# Autodesk Inventor assembly: MultiPassSCAN_outsideIn-DFMOD
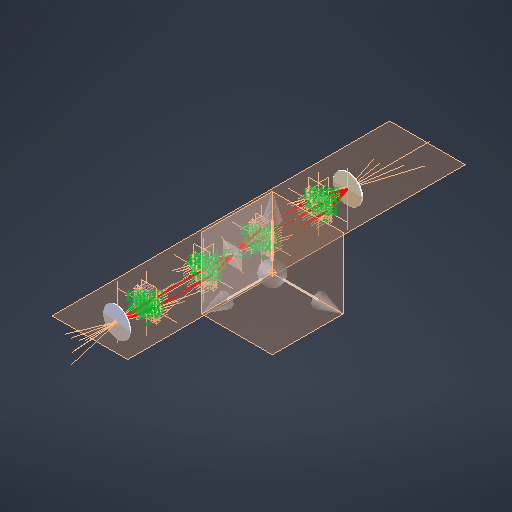
[picture p0: Inventor's stored thumbnail of the model, 512x512]
Saved by Autodesk Inventor 2026.1 (Build 301233000, 233)
## iProperties
Created: 2024-08-19
Part Number: MultiPassSCAN_outsideIn-DFMOD
Document SubType Name: Assembly
Designer: User
Author: User
## Documents named in this file (15)
- C:\Users\farin012\Downloads\fig4\fig4\MultiPassSCAN_outsideIn-DFMOD.iam
- C:\Users\farin012\Downloads\fig4\fig4\BB1-E02-Solidworks.ipt
- C:\Users\farin012\Downloads\fig4\fig4\LaserBeamEntry2.ipt
- C:\Users\farin012\Downloads\fig4\fig4\LoopPlane1.ipt
- C:\Users\farin012\Downloads\fig4\fig4\LA1608-AB-Solidworks\LA1608-AB-2LOOP_grid.ipt
- C:\Users\farin012\Downloads\fig4\fig4\LOOP1_COLL.ipt
- C:\Users\farin012\Downloads\fig4\fig4\LOOP1_COLL_PREDEF1.ipt
- C:\Users\farin012\Downloads\fig4\fig4\LOOP1_COLL_POSTDEF1.ipt
- C:\Users\farin012\Downloads\fig4\fig4\deflection_plane.ipt
- C:\Users\farin012\Downloads\fig4\fig4\LOOP1_COLL_PREDEF2.ipt
- C:\Users\farin012\Downloads\fig4\fig4\LOOP1_COLL_POSTDEF2.ipt
- C:\Users\farin012\Downloads\fig4\fig4\LOOP2_COLL_PREDEF1.ipt
- C:\Users\farin012\Downloads\fig4\fig4\LOOP2_COLL_POSTDEF1.ipt
- C:\Users\farin012\Downloads\fig4\fig4\LOOP2_COLL_PREDEF2.ipt
- C:\Users\farin012\Downloads\fig4\fig4\LOOP2_COLL_POSTDEF2.ipt
## Components (40 placed, 14 different names)
1. BB1-E02-Solidworks:1 — Mate:115, Mate:125, Mate:126, Mate:127, Angle:6, Mate:128, Mate:147
2. BB1-E02-Solidworks:2 — Angle:5, Mate:137, Mate:138
3. LaserBeamEntry2:16 — Mate:124, Flush:7
4. LoopPlane1:1 — Mate:113
5. LA1608-AB-2LOOP_grid:1 — Flush:3, Mate:124, Flush:7, Flush:8, Mate:129, Mate:145, Mate:147, Mate:148, Mate:172, Flush:164, Mate:173, Mate:174, Mate:175, Mate:176, Mate:177, Flush:165
6. LA1608-AB-2LOOP_grid:2 — Flush:2, Flush:9, Mate:130, Mate:145, Mate:146, Mate:149, Mate:154, Mate:155, Mate:156, Mate:169, Mate:170, Mate:171, Flush:163, Mate:178, Flush:166, Mate:179, Mate:180, Mate:193, Mate:194, Mate:195, Flush:171
7. LA1608-AB-2LOOP_grid:3 — Flush:5, Mate:137, Mate:151, Mate:152, Mate:160, Flush:160, Mate:161, Mate:162, Mate:163, Mate:164, Mate:165, Flush:161, Mate:184, Flush:168, Mate:185, Mate:186, Mate:187, Mate:188, Mate:189, Flush:169
8. LA1608-AB-2LOOP_grid:4 — Flush:4, Mate:146, Mate:150, Mate:152, Mate:159, Flush:159, Mate:166, Flush:162, Mate:167, Mate:168, Mate:181, Mate:182, Mate:183, Flush:167, Mate:190, Flush:170, Mate:191, Mate:192
9. LOOP1_COLL:1 — Mate:125, Mate:126
10. LOOP1_COLL:2 — Mate:127, Mate:128
11. LaserBeamEntry2:17 — Flush:8, Mate:129
12. LaserBeamEntry2:18 — Flush:9, Mate:130
13. LOOP1_COLL_PREDEF1:1 — Mate:155, Mate:156
14. LOOP1_COLL_POSTDEF1:1 — Mate:157, Mate:158
15. deflection_plane:1 — Mate:153, Mate:154, Flush:158, Mate:157, Mate:158
16. LaserBeamEntry2:19 — Mate:159, Flush:159
17. LaserBeamEntry2:20 — Mate:160, Flush:160
18. LOOP1_COLL_POSTDEF1:2 — Mate:161, Mate:162
19. LOOP1_COLL_POSTDEF1:3 — Mate:163, Mate:164
20. LaserBeamEntry2:21 — Mate:166, Flush:162
21. LaserBeamEntry2:22 — Mate:165, Flush:161
22. LOOP1_COLL_PREDEF2:1 — Mate:167, Mate:168
23. LOOP1_COLL_POSTDEF2:1 — Mate:169, Mate:170
24. LaserBeamEntry2:23 — Mate:172, Flush:164
25. LaserBeamEntry2:24 — Mate:171, Flush:163
26. LOOP2_COLL_PREDEF1:1 — Mate:173, Mate:174
27. LOOP2_COLL_PREDEF1:2 — Mate:175, Mate:176
28. LaserBeamEntry2:25 — Mate:177, Flush:165
29. LaserBeamEntry2:26 — Mate:178, Flush:166
30. LOOP2_COLL_PREDEF1:3 — Mate:179, Mate:180
31. LOOP2_COLL_POSTDEF1:1 — Mate:181, Mate:182
32. LaserBeamEntry2:27 — Mate:184, Flush:168
33. LaserBeamEntry2:28 — Mate:183, Flush:167
34. LOOP2_COLL_POSTDEF1:2 — Mate:185, Mate:186
35. LOOP2_COLL_PREDEF2:1 — Mate:187, Mate:188
36. LaserBeamEntry2:29 — Mate:189, Flush:169
37. LaserBeamEntry2:30 — Mate:190, Flush:170
38. LOOP2_COLL_PREDEF2:2 — Mate:191, Mate:192
39. LOOP2_COLL_POSTDEF2:1 — Mate:193, Mate:194
40. LaserBeamEntry2:31 — Mate:195, Flush:171
## Relationships (87: Mate 64, Flush 21, Angle 2)
- Mate:22
- Mate:23
- Mate:113: LoopPlane1:1
- Mate:115: BB1-E02-Solidworks:1
- Angle:5 (180 deg): BB1-E02-Solidworks:2
- Flush:2: LA1608-AB-2LOOP_grid:2
- Flush:3: LA1608-AB-2LOOP_grid:1
- Flush:4: LA1608-AB-2LOOP_grid:4
- Flush:5: LA1608-AB-2LOOP_grid:3
- Mate:124: LaserBeamEntry2:16 ↔ LA1608-AB-2LOOP_grid:1
- Flush:7: LaserBeamEntry2:16 ↔ LA1608-AB-2LOOP_grid:1
- Mate:125: BB1-E02-Solidworks:1 ↔ LOOP1_COLL:1
- Mate:126: BB1-E02-Solidworks:1 ↔ LOOP1_COLL:1
- Mate:127: BB1-E02-Solidworks:1 ↔ LOOP1_COLL:2
- Angle:6 (0 deg): BB1-E02-Solidworks:1
- Mate:128: BB1-E02-Solidworks:1 ↔ LOOP1_COLL:2
- Flush:8: LA1608-AB-2LOOP_grid:1 ↔ LaserBeamEntry2:17
- Mate:129: LA1608-AB-2LOOP_grid:1 ↔ LaserBeamEntry2:17
- Flush:9: LA1608-AB-2LOOP_grid:2 ↔ LaserBeamEntry2:18
- Mate:130: LA1608-AB-2LOOP_grid:2 ↔ LaserBeamEntry2:18
- Mate:137 (25 mm): BB1-E02-Solidworks:2 ↔ LA1608-AB-2LOOP_grid:3
- Mate:138: BB1-E02-Solidworks:2
- Mate:145 (-50 mm): LA1608-AB-2LOOP_grid:1 ↔ LA1608-AB-2LOOP_grid:2
- Mate:146 (50 mm): LA1608-AB-2LOOP_grid:2 ↔ LA1608-AB-2LOOP_grid:4
- Mate:147 (25 mm): BB1-E02-Solidworks:1 ↔ LA1608-AB-2LOOP_grid:1
- Mate:148: LA1608-AB-2LOOP_grid:1
- Mate:149: LA1608-AB-2LOOP_grid:2
- Mate:150: LA1608-AB-2LOOP_grid:4
- Mate:151: LA1608-AB-2LOOP_grid:3
- Mate:152 (-50 mm): LA1608-AB-2LOOP_grid:3 ↔ LA1608-AB-2LOOP_grid:4
- Mate:153: deflection_plane:1
- Mate:154 (25 mm): LA1608-AB-2LOOP_grid:2 ↔ deflection_plane:1
- Mate:155: LA1608-AB-2LOOP_grid:2 ↔ LOOP1_COLL_PREDEF1:1
- Mate:156: LA1608-AB-2LOOP_grid:2 ↔ LOOP1_COLL_PREDEF1:1
- Flush:158: deflection_plane:1
- Mate:157: LOOP1_COLL_POSTDEF1:1 ↔ deflection_plane:1
- Mate:158: LOOP1_COLL_POSTDEF1:1 ↔ deflection_plane:1
- Mate:159: LA1608-AB-2LOOP_grid:4 ↔ LaserBeamEntry2:19
- Flush:159: LA1608-AB-2LOOP_grid:4 ↔ LaserBeamEntry2:19
- Mate:160: LA1608-AB-2LOOP_grid:3 ↔ LaserBeamEntry2:20
- Flush:160: LA1608-AB-2LOOP_grid:3 ↔ LaserBeamEntry2:20
- Mate:161: LA1608-AB-2LOOP_grid:3 ↔ LOOP1_COLL_POSTDEF1:2
- Mate:162: LA1608-AB-2LOOP_grid:3 ↔ LOOP1_COLL_POSTDEF1:2
- Mate:163: LA1608-AB-2LOOP_grid:3 ↔ LOOP1_COLL_POSTDEF1:3
- Mate:164: LA1608-AB-2LOOP_grid:3 ↔ LOOP1_COLL_POSTDEF1:3
- Mate:165: LA1608-AB-2LOOP_grid:3 ↔ LaserBeamEntry2:22
- Flush:161: LA1608-AB-2LOOP_grid:3 ↔ LaserBeamEntry2:22
- Mate:166: LA1608-AB-2LOOP_grid:4 ↔ LaserBeamEntry2:21
- Flush:162: LA1608-AB-2LOOP_grid:4 ↔ LaserBeamEntry2:21
- Mate:167: LA1608-AB-2LOOP_grid:4 ↔ LOOP1_COLL_PREDEF2:1
- Mate:168: LA1608-AB-2LOOP_grid:4 ↔ LOOP1_COLL_PREDEF2:1
- Mate:169: LA1608-AB-2LOOP_grid:2 ↔ LOOP1_COLL_POSTDEF2:1
- Mate:170: LA1608-AB-2LOOP_grid:2 ↔ LOOP1_COLL_POSTDEF2:1
- Mate:171: LA1608-AB-2LOOP_grid:2 ↔ LaserBeamEntry2:24
- Flush:163: LA1608-AB-2LOOP_grid:2 ↔ LaserBeamEntry2:24
- Mate:172: LA1608-AB-2LOOP_grid:1 ↔ LaserBeamEntry2:23
- Flush:164: LA1608-AB-2LOOP_grid:1 ↔ LaserBeamEntry2:23
- Mate:173: LA1608-AB-2LOOP_grid:1 ↔ LOOP2_COLL_PREDEF1:1
- Mate:174: LA1608-AB-2LOOP_grid:1 ↔ LOOP2_COLL_PREDEF1:1
- Mate:175: LA1608-AB-2LOOP_grid:1 ↔ LOOP2_COLL_PREDEF1:2
- Mate:176: LA1608-AB-2LOOP_grid:1 ↔ LOOP2_COLL_PREDEF1:2
- Mate:177: LA1608-AB-2LOOP_grid:1 ↔ LaserBeamEntry2:25
- Flush:165: LA1608-AB-2LOOP_grid:1 ↔ LaserBeamEntry2:25
- Mate:178: LA1608-AB-2LOOP_grid:2 ↔ LaserBeamEntry2:26
- Flush:166: LA1608-AB-2LOOP_grid:2 ↔ LaserBeamEntry2:26
- Mate:179: LA1608-AB-2LOOP_grid:2 ↔ LOOP2_COLL_PREDEF1:3
- Mate:180: LA1608-AB-2LOOP_grid:2 ↔ LOOP2_COLL_PREDEF1:3
- Mate:181: LA1608-AB-2LOOP_grid:4 ↔ LOOP2_COLL_POSTDEF1:1
- Mate:182: LA1608-AB-2LOOP_grid:4 ↔ LOOP2_COLL_POSTDEF1:1
- Mate:183: LA1608-AB-2LOOP_grid:4 ↔ LaserBeamEntry2:28
- Flush:167: LA1608-AB-2LOOP_grid:4 ↔ LaserBeamEntry2:28
- Mate:184: LA1608-AB-2LOOP_grid:3 ↔ LaserBeamEntry2:27
- Flush:168: LA1608-AB-2LOOP_grid:3 ↔ LaserBeamEntry2:27
- Mate:185: LA1608-AB-2LOOP_grid:3 ↔ LOOP2_COLL_POSTDEF1:2
- Mate:186: LA1608-AB-2LOOP_grid:3 ↔ LOOP2_COLL_POSTDEF1:2
- Mate:187: LA1608-AB-2LOOP_grid:3 ↔ LOOP2_COLL_PREDEF2:1
- Mate:188: LA1608-AB-2LOOP_grid:3 ↔ LOOP2_COLL_PREDEF2:1
- Mate:189: LA1608-AB-2LOOP_grid:3 ↔ LaserBeamEntry2:29
- Flush:169: LA1608-AB-2LOOP_grid:3 ↔ LaserBeamEntry2:29
- Mate:190: LA1608-AB-2LOOP_grid:4 ↔ LaserBeamEntry2:30
- Flush:170: LA1608-AB-2LOOP_grid:4 ↔ LaserBeamEntry2:30
- Mate:191: LA1608-AB-2LOOP_grid:4 ↔ LOOP2_COLL_PREDEF2:2
- Mate:192: LA1608-AB-2LOOP_grid:4 ↔ LOOP2_COLL_PREDEF2:2
- Mate:193: LA1608-AB-2LOOP_grid:2 ↔ LOOP2_COLL_POSTDEF2:1
- Mate:194: LA1608-AB-2LOOP_grid:2 ↔ LOOP2_COLL_POSTDEF2:1
- Mate:195: LA1608-AB-2LOOP_grid:2 ↔ LaserBeamEntry2:31
- Flush:171: LA1608-AB-2LOOP_grid:2 ↔ LaserBeamEntry2:31
